# Autodesk Inventor assembly: brush assy
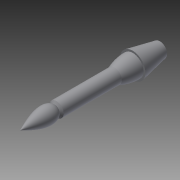
[picture p0: Inventor's stored thumbnail of the model, 180x180]
Saved by Autodesk Inventor 2013 SP2 (Build 170200200, 200)
## iProperties
Created: 2017-05-30
Part Number: brush assy
Document SubType Name: Assembly
Designer: Herman de Vries
Author: Herman de Vries
## Documents named in this file (4)
- C:\Users\hdv\Dropbox\Projects\Inventor\PaintBot_3\Brush holder\brush assy.iam
- C:\Users\hdv\Dropbox\Projects\Inventor\PaintBot_3\Brush holder\brush - cut.ipt
- C:\Users\hdv\Dropbox\Projects\Inventor\PaintBot_3\Brush holder\brush fitting partb.ipt
- C:\Users\hdv\Dropbox\Projects\Inventor\PaintBot_3\Brush holder\brush fitting.ipt
## Components (3 placed, 3 different names)
1. brush - cut:1 — Insert:1
2. brush fitting partb:1 — Insert:2
3. brush fitting:1 — Insert:1, Insert:2
## Relationships (2: Insert 2)
- Insert:1: brush - cut:1 ↔ brush fitting:1
- Insert:2: brush fitting partb:1 ↔ brush fitting:1
